# Autodesk Inventor assembly: Interface_assembly
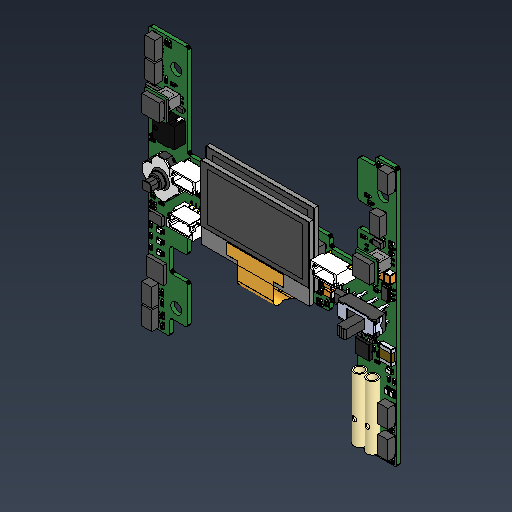
[picture p0: Inventor's stored thumbnail of the model, 512x512]
Saved by Autodesk Inventor 2026.2 (Build 302298010, 298A)
## iProperties
Created: 2026-05-10
Part Number: Interface_assembly
Document SubType Name: Assembly
Designer: szymo
Author: szymo
## Documents named in this file (4)
- D:\tech\robotyka\robots\evangelion-turbo\3DP\Interface_assembly.iam
- D:\tech\robotyka\robots\evangelion-turbo\inventor-project\PCBMain\PCBMain\PCBMain.ipt
- D:\tech\robotyka\robots\evangelion-turbo\inventor-project\PCBIr\PCBIr\PCBIr.ipt
- D:\tech\robotyka\robots\evangelion-turbo\inventor-project\0.96 oled\0.96 oled\0.96 oled.ipt
## Components (4 placed, 3 different names)
1. PCBMain:1 — Flush:1, Flush:2, Mate:1, Mate:2, Flush:3, Flush:4, Flush:5, Mate:3, Flush:6, Flush:7
2. PCBIr:1 — Flush:1, Flush:2, Mate:1
3. 0.96 oled:1 — Flush:5, Mate:3, Flush:6, Flush:7
4. PCBIr:2 — Mate:2, Flush:3, Flush:4
## Relationships (10: Flush 7, Mate 3)
- Flush:1 (-0.051 mm): PCBMain:1 ↔ PCBIr:1
- Flush:2 (0.1015 mm): PCBMain:1 ↔ PCBIr:1
- Mate:1: PCBMain:1 ↔ PCBIr:1
- Mate:2: PCBMain:1 ↔ PCBIr:2
- Flush:3 (0.051 mm): PCBMain:1 ↔ PCBIr:2
- Flush:4 (0.1015 mm): PCBMain:1 ↔ PCBIr:2
- Flush:5: PCBMain:1 ↔ 0.96 oled:1
- Mate:3 (0.5 mm): PCBMain:1 ↔ 0.96 oled:1
- Flush:6: PCBMain:1 ↔ 0.96 oled:1
- Flush:7 (-2.5 mm): PCBMain:1 ↔ 0.96 oled:1
